# Autodesk Inventor assembly: akkufach
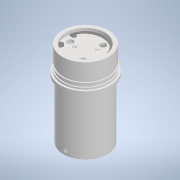
[picture p0: Inventor's stored thumbnail of the model, 180x180]
Saved by Autodesk Inventor 2020.2 (Build 242310000, 310)
## iProperties
Created: 2020-11-11
Part Number: akkufach
Document SubType Name: Assembly
Designer: g.schardt
Author: g.schardt
## Documents named in this file (4)
- C:\Users\g.schardt\Inventor\Tauchlampe\akkufach.iam
- C:\Users\g.schardt\Inventor\Tauchlampe\akkufach_deckel.ipt
- C:\Users\g.schardt\Documents\Inventor\Content Center Files\R2020\de-DE\DIN 472(2)\DIN 472 - 40x1,75.ipt
- C:\Users\g.schardt\Inventor\Tauchlampe\akkufach_.ipt
## Components (3 placed, 3 different names)
1. akkufach_:1 — Passend:1, Fluchtend:1, Passend:2, Fluchtend:3, Einfügen:1
2. akkufach_deckel:1 — Passend:2, Fluchtend:3
3. DIN 472 40x1,75:1 — Einfügen:1
## Relationships (5: Mate 2, Flush 2, Insert 1)
- Passend:1 [Mate]: akkufach_:1
- Fluchtend:1 [Flush] (-45 mm): akkufach_:1
- Passend:2 [Mate]: akkufach_:1 ↔ akkufach_deckel:1
- Fluchtend:3 [Flush]: akkufach_:1 ↔ akkufach_deckel:1
- Einfügen:1 [Insert]: akkufach_:1 ↔ DIN 472 40x1,75:1
